# Autodesk Inventor assembly: Copleto1
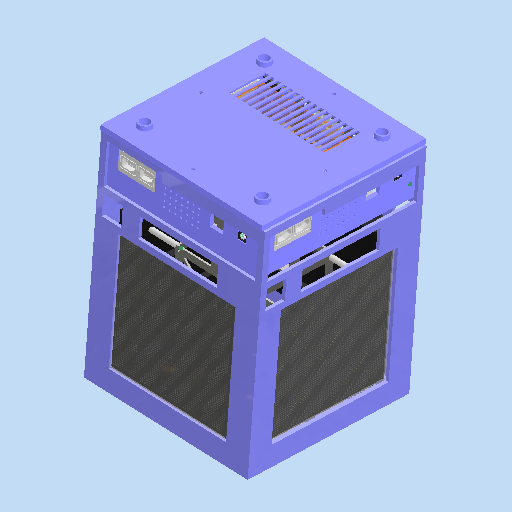
[picture p0: Inventor's stored thumbnail of the model, 512x512]
Saved by Autodesk Inventor 2027 (Build 310192000, 192)
## iProperties
Created: 2026-10-07
Part Number: Copleto1
Document SubType Name: Weldment
Designer: alex
Weld Material: Welded Aluminum-6061
Author: alex
## Documents named in this file (3)
- C:\Users\alex\Documents\BocetoDigital\Copleto1.iam
- C:\Users\alex\Documents\BocetoDigital\Parte Medio\ParteMeida.iam
- C:\Users\alex\Documents\BocetoDigital\Parte Superior\Tapa superior.ipt
## Components (2 placed, 2 different names)
1. Tapa superior:1 — Coincidencia:1, Coincidencia:2, Coincidencia:3
2. ParteMeida:1 [sub-assembly] — Coincidencia:1, Coincidencia:2, Coincidencia:3
## Relationships (3: Mate 3)
- Coincidencia:1 [Mate]: Tapa superior:1 ↔ ParteMeida:1
- Coincidencia:2 [Mate]: Tapa superior:1 ↔ ParteMeida:1
- Coincidencia:3 [Mate]: Tapa superior:1 ↔ ParteMeida:1
